# Autodesk Inventor assembly: МД.001.1000 - Захват
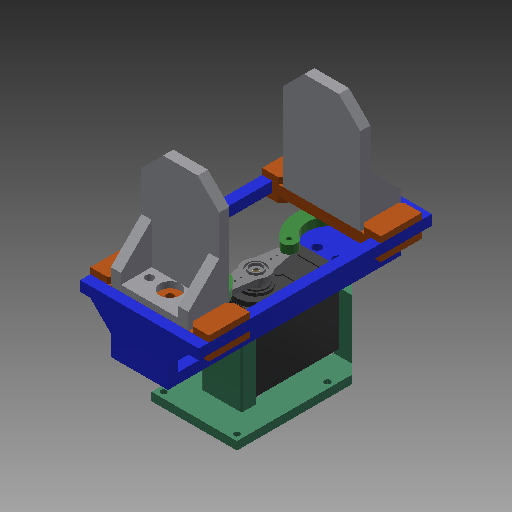
[picture p0: Inventor's stored thumbnail of the model, 512x512]
Saved by Autodesk Inventor 2019 (Build 230136000, 136)
## iProperties
Created: 2019-12-30
Part Number: МД.001.1000 - Захват
Material: Типовые
Document SubType Name: Assembly
Designer: Петров Иван
Author: Петров Иван
## Documents named in this file (8)
- E:\IVAN\Ivan_desktop\GitHub\Arm_manip\hardware\МД.001.1000 - Захват.iam
- E:\IVAN\Ivan_desktop\GitHub\Arm_manip\hardware\МД.001.1001 - Опора захвата.ipt
- E:\IVAN\Ivan_desktop\GitHub\Arm_manip\hardware\Standart_things\tower prone.ipt
- E:\IVAN\Ivan_desktop\GitHub\Arm_manip\hardware\МД.001.1002 - Станина.ipt
- E:\IVAN\Ivan_desktop\inventor\Models\Models\Motors and servo\Servo\tower-pro-mg-995-analog-servo-1.snapshot.8\TOWER PRO MG-995, ANALOG SERVO, HORN.ipt
- E:\IVAN\Ivan_desktop\GitHub\Arm_manip\hardware\МД.001.1003 - Салазка.ipt
- E:\IVAN\Ivan_desktop\GitHub\Arm_manip\hardware\МД.001.1004 - Скоба.ipt
- E:\IVAN\Ivan_desktop\GitHub\Arm_manip\hardware\МД.001.1005 - Прихват.ipt
## Components (10 placed, 7 different names)
1. МД.001.1001 - Опора захвата:1 — Совмещение:1, Совмещение:2, Совмещение:3, Совмещение:5
2. tower prone:1 — Совмещение:1, Совмещение:2, Совмещение:3, Совмещение:4, Совмещение:6, Совмещение:7, Совмещение:8
3. МД.001.1002 - Станина:1 — Совмещение:4, Совмещение:5, Совмещение:6, Угол:1, Совмещение:9, Совмещение:10, Ограничение смещения, Совмещение:12, Ограничение смещения 2, Совмещение:14
4. TOWER PRO MG-995, ANALOG SERVO, HORN:1 — Совмещение:7, Совмещение:8, Угол:1, Совмещение:15, Совмещение:16, Совмещение:18, Совмещение:19
5. МД.001.1003 - Салазка:1 — Совмещение:9, Совмещение:10, Ограничение смещения, Совмещение:20, Совмещение:24, Совмещение:25, Совмещение:26
6. МД.001.1003 - Салазка:2 — Совмещение:12, Ограничение смещения 2, Совмещение:14, Совмещение:17, Совмещение:21, Совмещение:22, Совмещение:23
7. МД.001.1004 - Скоба:1 — Совмещение:15, Совмещение:16, Совмещение:17
8. МД.001.1004 - Скоба:2 — Совмещение:18, Совмещение:19, Совмещение:20
9. МД.001.1005 - Прихват:1 — Совмещение:21, Совмещение:22, Совмещение:23
10. МД.001.1005 - Прихват:2 — Совмещение:24, Совмещение:25, Совмещение:26
## Relationships (27: Mate 26, Angle 1)
- Совмещение:1 [Mate]: МД.001.1001 - Опора захвата:1 ↔ tower prone:1
- Совмещение:2 [Mate]: МД.001.1001 - Опора захвата:1 ↔ tower prone:1
- Совмещение:3 [Mate]: МД.001.1001 - Опора захвата:1 ↔ tower prone:1
- Совмещение:4 [Mate]: tower prone:1 ↔ МД.001.1002 - Станина:1
- Совмещение:5 [Mate]: МД.001.1001 - Опора захвата:1 ↔ МД.001.1002 - Станина:1
- Совмещение:6 [Mate]: tower prone:1 ↔ МД.001.1002 - Станина:1
- Совмещение:7 [Mate]: tower prone:1 ↔ TOWER PRO MG-995, ANALOG SERVO, HORN:1
- Совмещение:8 [Mate]: tower prone:1 ↔ TOWER PRO MG-995, ANALOG SERVO, HORN:1
- Угол:1 [Angle] (0 deg): МД.001.1002 - Станина:1 ↔ TOWER PRO MG-995, ANALOG SERVO, HORN:1
- Совмещение:9 [Mate]: МД.001.1002 - Станина:1 ↔ МД.001.1003 - Салазка:1
- Совмещение:10 [Mate]: МД.001.1002 - Станина:1 ↔ МД.001.1003 - Салазка:1
- Ограничение смещения [Mate]: МД.001.1002 - Станина:1 ↔ МД.001.1003 - Салазка:1
- Совмещение:12 [Mate]: МД.001.1002 - Станина:1 ↔ МД.001.1003 - Салазка:2
- Ограничение смещения 2 [Mate]: МД.001.1002 - Станина:1 ↔ МД.001.1003 - Салазка:2
- Совмещение:14 [Mate]: МД.001.1002 - Станина:1 ↔ МД.001.1003 - Салазка:2
- Совмещение:15 [Mate]: TOWER PRO MG-995, ANALOG SERVO, HORN:1 ↔ МД.001.1004 - Скоба:1
- Совмещение:16 [Mate]: TOWER PRO MG-995, ANALOG SERVO, HORN:1 ↔ МД.001.1004 - Скоба:1
- Совмещение:17 [Mate]: МД.001.1003 - Салазка:2 ↔ МД.001.1004 - Скоба:1
- Совмещение:18 [Mate]: TOWER PRO MG-995, ANALOG SERVO, HORN:1 ↔ МД.001.1004 - Скоба:2
- Совмещение:19 [Mate]: TOWER PRO MG-995, ANALOG SERVO, HORN:1 ↔ МД.001.1004 - Скоба:2
- Совмещение:20 [Mate]: МД.001.1003 - Салазка:1 ↔ МД.001.1004 - Скоба:2
- Совмещение:21 [Mate]: МД.001.1003 - Салазка:2 ↔ МД.001.1005 - Прихват:1
- Совмещение:22 [Mate]: МД.001.1003 - Салазка:2 ↔ МД.001.1005 - Прихват:1
- Совмещение:23 [Mate]: МД.001.1003 - Салазка:2 ↔ МД.001.1005 - Прихват:1
- Совмещение:24 [Mate]: МД.001.1003 - Салазка:1 ↔ МД.001.1005 - Прихват:2
- Совмещение:25 [Mate]: МД.001.1003 - Салазка:1 ↔ МД.001.1005 - Прихват:2
- Совмещение:26 [Mate]: МД.001.1003 - Салазка:1 ↔ МД.001.1005 - Прихват:2
